# Autodesk Inventor assembly: MX-28T_R+idle.ipt_MIR
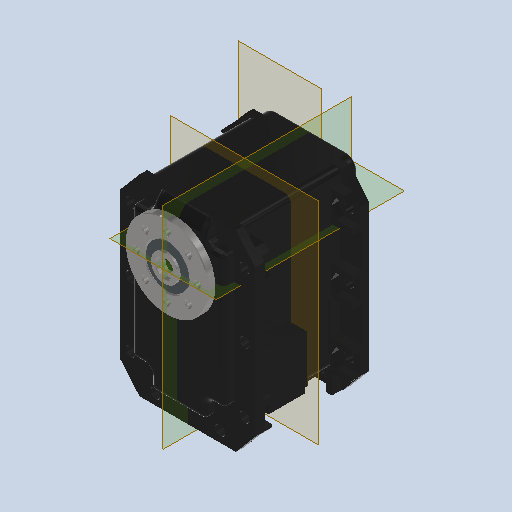
[picture p0: Inventor's stored thumbnail of the model, 512x512]
Saved by Autodesk Inventor 2024.3 (Build 283343000, 343)
## iProperties
Created: 2022-08-09
Part Number: MX-28T_R+idle.ipt_MIR
Document SubType Name: Assembly
Designer: 구지현
Mass: 83 g
Surface Area: 131.328 cm^2
Volume: 44.8383 cm^3
Author: 박지훈
## Documents named in this file (3)
- C:\Users\구지현\Documents\카카오톡 받은 파일\Hardware\ROBOTIS(Inventor 2024 ver.)\다이나믹셀\MX-28T_R+idle.ipt_MIR.iam
- C:\Users\구지현\Documents\카카오톡 받은 파일\Hardware\ROBOTIS(Inventor 2024 ver.)\아이들러\28아이들러_MIR.iam
- C:\Users\구지현\Documents\카카오톡 받은 파일\Hardware\ROBOTIS(Inventor 2024 ver.)\다이나믹셀\MX-28T_R_MIR.ipt
## Components (2 placed, 2 different names)
1. 28아이들러_MIR:1 [sub-assembly] — 삽입:1
2. MX-28T_R_MIR:1 — 삽입:1
## Relationships (1: Insert 1)
- 삽입:1 [Insert] (0.1 mm): 28아이들러_MIR:1 ↔ MX-28T_R_MIR:1
